# Autodesk Inventor assembly: aa_Pallet_BTP_template
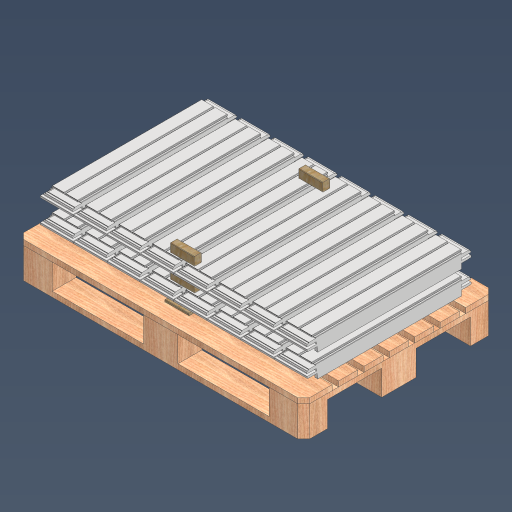
[picture p0: Inventor's stored thumbnail of the model, 512x512]
Saved by Autodesk Inventor 2023.2 (Build 272271030, 271C)
## iProperties
Category: Moduł
RuleStatus: InUse
Created: 2024-08-05
Part Number: aa_Pallet_BTP_template
Document SubType Name: Assembly
Designer: Robert Łapiński
Stock Number: aa_Pallet_BTP_template
Mass: 62965 g
Surface Area: 68416.5 cm^2
Volume: 83700.5 cm^3
Density: 0.752266 g/cm^3
Magazyn: False
Producent: Hitmark Sp. z o. o.
DocNumber: Zespół1.iam
Folder: .\
VDS_Category: Inżynierski
Technologia_1: Brak
Technologia_2: Brak
Technologia_3: Brak
Technologia_4: Brak
Author: Robert Łapiński
## Documents named in this file (6)
- C:\Users\ROBERT\Desktop\VELUX\Komponenty\Velux Pallets\aa_Pallet_BTP_template.iam
- C:\Users\ROBERT\Desktop\VELUX\Komponenty\Przekladki i palety\Paleta europejska\EP_800x1200x150.ipt
- C:\Users\ROBERT\Desktop\VELUX\Komponenty\Przekladki i palety\PAL_EUR_.ipt
- C:\Users\ROBERT\Desktop\VELUX\Komponenty\Przekladki i palety\S1_.ipt
- C:\Users\ROBERT\Desktop\VELUX\Komponenty\Przekladki i palety\S3_.ipt
- C:\Users\ROBERT\Desktop\VELUX\Komponenty\Velux Models_BTP\Models\GDL P1 Bottom Sash MK.ipt
## Components (23 placed, 4 different names)
1. EP_800x1200x150:1 — Mate:1, Flush:1, Angle:3
2. S1_:1
3. S1_:2
4. GDL P1 Bottom Sash MK:1 — Angle:1
5. GDL P1 Bottom Sash MK:2
6. GDL P1 Bottom Sash MK:3
7. GDL P1 Bottom Sash MK:4
8. GDL P1 Bottom Sash MK:5
9. GDL P1 Bottom Sash MK:6
10. GDL P1 Bottom Sash MK:7
11. GDL P1 Bottom Sash MK:8
12. GDL P1 Bottom Sash MK:9
13. GDL P1 Bottom Sash MK:10
14. GDL P1 Bottom Sash MK:11
15. GDL P1 Bottom Sash MK:12
16. GDL P1 Bottom Sash MK:13
17. GDL P1 Bottom Sash MK:14
18. GDL P1 Bottom Sash MK:15
19. GDL P1 Bottom Sash MK:16
20. S3_:1 — Angle:2
21. S3_:2
22. S3_:3
23. S3_:4
## Component patterns: Szyk_Vert_Comp:1 (2 elements), Szyk_Vert_Spacer:1 (2 elements), Szyk_First_Spacer:1 (2 elements), First_Layer_Comp 1:1 (8 elements), Component Pattern 1:2 (8 elements), First_Layer_Spacer:1 (2 elements), Component Pattern 2:2 (2 elements)
## Relationships (5: Angle 3, Mate 1, Flush 1)
- Angle:1 (0 deg): GDL P1 Bottom Sash MK:1
- Angle:2 (0 deg): S3_:1
- Mate:1: EP_800x1200x150:1
- Flush:1: EP_800x1200x150:1
- Angle:3 (0 deg): EP_800x1200x150:1
## Named parameters: n_Comp_Z_dist = 2000 mm, n_Comp_X_dist = 140.3 mm, n_Comp_X = 8, n_Spacer_X_dist = 100 mm, n_Spacer_Z_dist = 538.7 mm, n_Spacer_X = 1, n_Spacer_Z = 2, n_Comp_Y_dist = 97.4 mm, n_Comp_Y = 2, n_Spacer_Y_dist = 97.4 mm, n_Spacer_Y = 2, FirstSpacerGap = 640 mm, PalletAngle = 0 deg
